# Autodesk Inventor assembly: assembly
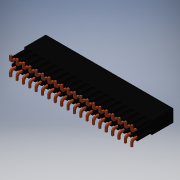
[picture p0: Inventor's stored thumbnail of the model, 180x180]
Saved by Autodesk Inventor 2016 (Build 200138000, 138)
## iProperties
Created: 2016-07-25
Part Number: assembly
Document SubType Name: Assembly
Designer: Jonathan
Author: Jonathan
## Documents named in this file (5)
- C:\Users\Jonathan\Documents\Projects\mppcInterface\4-channel\mppcInterface\cad\connector\SMT GPIO Female Header 2x20\assembly.iam
- C:\Users\Jonathan\Documents\Projects\mppcInterface\4-channel\mppcInterface\cad\connector\SMT GPIO Female Header 2x20\body.ipt
- C:\Users\Jonathan\Documents\Projects\mppcInterface\4-channel\mppcInterface\cad\connector\SMT GPIO Female Header 2x20\pins.ipt
- C:\Users\Jonathan\Documents\Projects\mppcInterface\4-channel\mppcInterface\cad\connector\SMT GPIO Female Header 2x20\body_MIR.ipt
- C:\Users\Jonathan\Documents\Projects\mppcInterface\4-channel\mppcInterface\cad\connector\SMT GPIO Female Header 2x20\pins_MIR.ipt
## Components (80 placed, 4 different names)
1. pins:1 — Mate:1, Mate:2, Flush:1
2. body:1 — Mate:1, Mate:2, Flush:1
3. pins:2
4. body:2
5. pins:3
6. body:3
7. pins:4
8. body:4
9. pins:5
10. body:5
11. pins:6
12. body:6
13. pins:7
14. body:7
15. pins:8
16. body:8
17. pins:9
18. body:9
19. pins:10
20. body:10
21. pins:11
22. body:11
23. pins:12
24. body:12
25. pins:13
26. body:13
27. pins:14
28. body:14
29. pins:15
30. body:15
31. pins:16
32. body:16
33. pins:17
34. body:17
35. pins:18
36. body:18
37. pins:19
38. body:19
39. pins:20
40. body:20
41. pins_MIR:1 — Flush:2, Mate:3, Mate:4
42. body_MIR:1 — Flush:2, Mate:3, Mate:4
43. pins_MIR:2
44. body_MIR:2
45. pins_MIR:3
46. body_MIR:3
47. pins_MIR:4
48. body_MIR:4
49. pins_MIR:5
50. body_MIR:5
51. pins_MIR:6
52. body_MIR:6
53. pins_MIR:7
54. body_MIR:7
55. pins_MIR:8
56. body_MIR:8
57. pins_MIR:9
58. body_MIR:9
59. pins_MIR:10
60. body_MIR:10
61. pins_MIR:11
62. body_MIR:11
63. pins_MIR:12
64. body_MIR:12
65. pins_MIR:13
66. body_MIR:13
67. pins_MIR:14
68. body_MIR:14
69. pins_MIR:15
70. body_MIR:15
71. pins_MIR:16
72. body_MIR:16
73. pins_MIR:17
74. body_MIR:17
75. pins_MIR:18
76. body_MIR:18
77. pins_MIR:19
78. body_MIR:19
79. pins_MIR:20
80. body_MIR:20
## Component patterns: (20 elements, first: pins:1 + body:1), (20 elements, first: pins_MIR:1 + body_MIR:1)
## Relationships (6: Mate 4, Flush 2)
- Mate:1: pins:1 ↔ body:1
- Mate:2: pins:1 ↔ body:1
- Flush:1 (-2 mm): pins:1 ↔ body:1
- Flush:2 (-2 mm): pins_MIR:1 ↔ body_MIR:1
- Mate:3: pins_MIR:1 ↔ body_MIR:1
- Mate:4: pins_MIR:1 ↔ body_MIR:1
